# Autodesk Inventor assembly: SwitchWMount
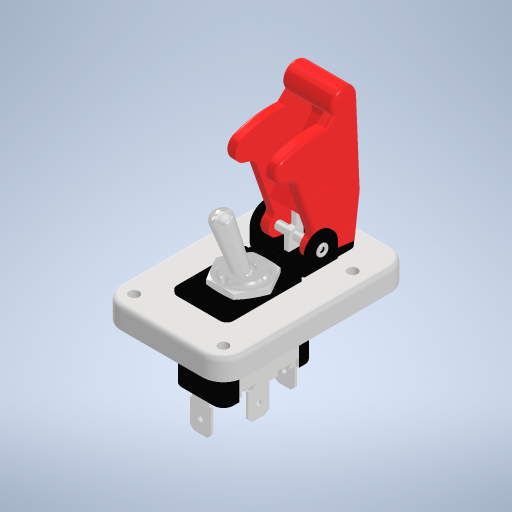
[picture p0: Inventor's stored thumbnail of the model, 512x512]
Saved by Autodesk Inventor 2024 (Build 280153000, 153)
## iProperties
Created: 2023-04-06
Part Number: SwitchWMount
Document SubType Name: Assembly
Designer: richb366163
Author: richb366163
## Documents named in this file (3)
- C:\Users\18179\Desktop\RoboBoatV2\SwitchWMount.iam
- C:\Users\18179\Desktop\RoboBoatV2\SwitchHolder.ipt
- C:\Users\18179\Desktop\RoboBoatV2\Switch With Guard.iam
## Components (2 placed, 2 different names)
1. SwitchHolder:1 — Mate:1, Mate:2
2. Switch With Guard:1 [sub-assembly] — Mate:1, Mate:2
## Relationships (2: Mate 2)
- Mate:1: SwitchHolder:1 ↔ Switch With Guard:1
- Mate:2: SwitchHolder:1 ↔ Switch With Guard:1
